# Autodesk Inventor assembly: Assembly1
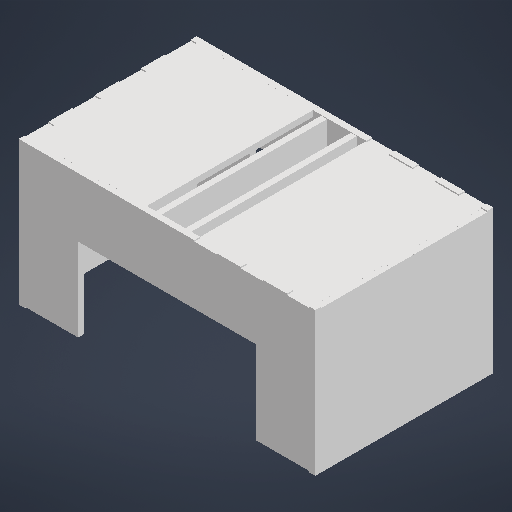
[picture p0: Inventor's stored thumbnail of the model, 512x512]
Saved by Autodesk Inventor 2027.1 (Build 311270010, 270A)
## iProperties
Created: 2026-10-07
Part Number: Assembly1
Document SubType Name: Assembly
Designer: daniel
Author: daniel
## Documents named in this file (5)
- C:\Users\danda\Desktop\Design 1\Project\CAD\box\Assembly1.iam
- C:\Users\danda\Desktop\Design 1\Project\CAD\box\Part2.ipt
- C:\Users\danda\Desktop\Design 1\Project\CAD\box\Part1.ipt
- C:\Users\danda\Desktop\Design 1\Project\CAD\box\Part3.ipt
- C:\Users\danda\Desktop\Design 1\Project\CAD\box\part4.ipt
## Components (9 placed, 4 different names)
1. Part2:1 — Mate:1, Flush:1, Mate:2, Mate:6, Mate:7, Flush:3, Mate:19
2. Part1:1 — Mate:1, Flush:1, Mate:2, Mate:3, Mate:4, Flush:2, Mate:8, Mate:9, Mate:10, Mate:15, Mate:18, Mate:21
3. Part2:2 — Mate:3, Mate:4, Flush:2, Mate:5, Mate:20, Mate:22
4. Part1:2 — Mate:5, Mate:6, Mate:7, Flush:3, Mate:11, Mate:12, Mate:13, Mate:14, Mate:16, Mate:17
5. Part3:1 — Mate:14, Mate:15, Mate:16
6. Part3:2 — Mate:11, Mate:12, Mate:13
7. Part3:3 — Mate:8, Mate:9, Mate:10
8. part4:1 — Mate:20, Mate:21, Mate:22
9. part4:2 — Mate:17, Mate:18, Mate:19
## Relationships (25: Mate 22, Flush 3)
- Mate:1: Part2:1 ↔ Part1:1
- Flush:1: Part2:1 ↔ Part1:1
- Mate:2: Part2:1 ↔ Part1:1
- Mate:3: Part1:1 ↔ Part2:2
- Mate:4: Part1:1 ↔ Part2:2
- Flush:2: Part1:1 ↔ Part2:2
- Mate:5: Part2:2 ↔ Part1:2
- Mate:6: Part2:1 ↔ Part1:2
- Mate:7: Part2:1 ↔ Part1:2
- Flush:3: Part2:1 ↔ Part1:2
- Mate:8: Part1:1 ↔ Part3:3
- Mate:9: Part1:1 ↔ Part3:3
- Mate:10: Part1:1 ↔ Part3:3
- Mate:11: Part1:2 ↔ Part3:2
- Mate:12: Part1:2 ↔ Part3:2
- Mate:13: Part1:2 ↔ Part3:2
- Mate:14: Part1:2 ↔ Part3:1
- Mate:15: Part1:1 ↔ Part3:1
- Mate:16: Part1:2 ↔ Part3:1
- Mate:17: Part1:2 ↔ part4:2
- Mate:18: Part1:1 ↔ part4:2
- Mate:19: Part2:1 ↔ part4:2
- Mate:20: Part2:2 ↔ part4:1
- Mate:21: Part1:1 ↔ part4:1
- Mate:22: Part2:2 ↔ part4:1
